# Autodesk Inventor assembly: ECoG holder_2p1_3p0
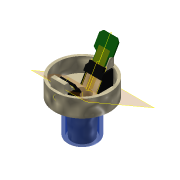
[picture p0: Inventor's stored thumbnail of the model, 180x180]
Saved by Autodesk Inventor 2014 (Build 180170000, 170)
## iProperties
Created: 2016-08-28
Part Number: ECoG holder_2p1_3p0
Document SubType Name: Assembly
Designer: Camilo
Author: Camilo
## Documents named in this file (8)
- Z:\Github\AgingTests\3D parts\ECoG holder_2p0\ECoG holder_2p1_3p0.iam
- Z:\Github\AgingTests\3D parts\ECoG holder\flaskPort_3p0.ipt
- Z:\Github\AgingTests\3D parts\ECoG holder_2p0\ECoG_holder_3p0.ipt
- Z:\Github\AgingTests\3D parts\ECoG holder_2p0\32ch_ECoG_assembled_3p0.iam
- Z:\Github\AgingTests\3D parts\ECoG holder_2p0\PTFEFilter_clamp_3p0.ipt
- Z:\Github\AgingTests\3D parts\ECoG holder_2p0\spaceFiller_3p0.ipt
- Z:\Github\AgingTests\3D parts\ECoG holder_2p0\spaceFiller_MIR1_3p0.ipt
- Z:\Github\AgingTests\3D parts\ECoG holder_2p0\PTFEFilter_clamp_MIR_3p0.ipt
## Components (7 placed, 7 different names)
1. flaskPort_3p0:1 — Mate:2, Flush:3, Mate:1, Flush:4
2. ECoG_holder_3p0:1 — Flush:4, Flush:5, Mate:4, Mate:3, Flush:7, Flush:6, Flush:9, Flush:8
3. 32ch_ECoG_assembled_3p0:1 [sub-assembly] — Flush:5, Mate:4, Mate:3
4. PTFEFilter_clamp_3p0:1 — Flush:7, Flush:6
5. spaceFiller_3p0:1 — Flush:9, Flush:8
6. spaceFiller_MIR1_3p0:1
7. PTFEFilter_clamp_MIR_3p0:1
## Relationships (11: Flush 7, Mate 4)
- Mate:2: flaskPort_3p0:1
- Flush:3: flaskPort_3p0:1
- Mate:1: flaskPort_3p0:1
- Flush:4: flaskPort_3p0:1 ↔ ECoG_holder_3p0:1
- Flush:5: ECoG_holder_3p0:1 ↔ 32ch_ECoG_assembled_3p0:1
- Mate:4: ECoG_holder_3p0:1 ↔ 32ch_ECoG_assembled_3p0:1
- Mate:3: ECoG_holder_3p0:1 ↔ 32ch_ECoG_assembled_3p0:1
- Flush:7: ECoG_holder_3p0:1 ↔ PTFEFilter_clamp_3p0:1
- Flush:6: ECoG_holder_3p0:1 ↔ PTFEFilter_clamp_3p0:1
- Flush:9: ECoG_holder_3p0:1 ↔ spaceFiller_3p0:1
- Flush:8: ECoG_holder_3p0:1 ↔ spaceFiller_3p0:1
